# Autodesk Inventor assembly: manipulator
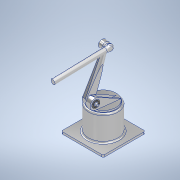
[picture p0: Inventor's stored thumbnail of the model, 180x180]
Saved by Autodesk Inventor 2022.2 (Build 262287010, 287A)
## iProperties
Created: 2022-04-10
Part Number: manipulator
Document SubType Name: Assembly
Designer: stasi
Author: stasi
## Documents named in this file (10)
- D:\stuff\P G\sem6\KPMiR\proj\kpmir\INVENTOR\manipulator.iam
- D:\stuff\P G\sem6\KPMiR\proj\kpmir\INVENTOR\C0.ipt
- D:\stuff\P G\sem6\KPMiR\proj\kpmir\INVENTOR\C1.ipt
- D:\stuff\P G\sem6\KPMiR\proj\kpmir\INVENTOR\C2.ipt
- D:\stuff\P G\sem6\KPMiR\proj\kpmir\INVENTOR\C3.ipt
- D:\stuff\P G\sem6\KPMiR\proj\kpmir\INVENTOR\manipulator\Design Accelerator\Bearing R11.iam
- D:\stuff\P G\sem6\KPMiR\proj\kpmir\INVENTOR\manipulator\Design Accelerator\Bearing R1v32.iam
- D:\stuff\P G\sem6\KPMiR\proj\kpmir\INVENTOR\manipulator\Design Accelerator\Bearing R24.iam
- D:\stuff\P G\sem6\KPMiR\proj\kpmir\INVENTOR\manipulator\Design Accelerator\Bearing R25.iam
- D:\stuff\P G\sem6\KPMiR\proj\kpmir\INVENTOR\manipulator\Design Accelerator\Bearing R2v21.iam
## Components (9 placed, 9 different names)
1. C0:1 — Flush:9, Flush:10, Flush:15, Mate:5, R0 AXIS
2. C1:1 — R1 AXIS, Flush:11, Mate:1, Flush:12, Mate:2, R0 AXIS
3. C2:1 — R1 AXIS, Flush:14, Mate:4, R2 AXIS, Flush:16
4. C3:1 — R2 AXIS, Mate:6
5. Bearing R1:1 [sub-assembly] — Flush:11, Mate:1
6. Bearing R1v2:1 [sub-assembly] — Flush:12, Mate:2
7. Bearing R2:1 [sub-assembly] — Flush:16, Mate:6
8. Bearing R2v2:1 [sub-assembly] — Flush:14, Mate:4
9. Bearing R0:1 [sub-assembly] — Flush:15, Mate:5
## Relationships (15: Flush 7, Mate 5, RevoluteJoint 3)
- Flush:9 (10 mm): C0:1
- R1 AXIS [RevoluteJoint]: C1:1 ↔ C2:1
- Flush:10: C0:1
- Flush:11: C1:1 ↔ Bearing R1:1
- Mate:1: C1:1 ↔ Bearing R1:1
- Flush:12: C1:1 ↔ Bearing R1v2:1
- Mate:2: C1:1 ↔ Bearing R1v2:1
- Flush:14: C2:1 ↔ Bearing R2v2:1
- Mate:4: C2:1 ↔ Bearing R2v2:1
- Flush:15: C0:1 ↔ Bearing R0:1
- Mate:5: C0:1 ↔ Bearing R0:1
- R0 AXIS [RevoluteJoint]: C0:1 ↔ C1:1
- R2 AXIS [RevoluteJoint]: C2:1 ↔ C3:1
- Flush:16: C2:1 ↔ Bearing R2:1
- Mate:6: C3:1 ↔ Bearing R2:1
